# Autodesk Inventor assembly: крепление
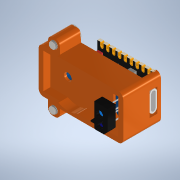
[picture p0: Inventor's stored thumbnail of the model, 180x180]
Saved by Autodesk Inventor 2022 (Build 260153000, 153)
## iProperties
Created: 2025-02-02
Part Number: крепление
Document SubType Name: Assembly
Designer: Admin
Author: Admin
## Documents named in this file (5)
- G:\машина\крепление.iam
- G:\машина\крепл. датчк.1.ipt
- G:\машина\ESP32S3 Super Mini.ipt
- G:\машина\Screw GB_T 13806.1-1992 B M3 x 10.ipt
- G:\машина\TCRT5000.iam
## Components (5 placed, 4 different names)
1. крепл. датчк.1:1 — Совмещение:7
2. ESP32S3 Super Mini:1
3. Screw GB/T 13806.1-1992 Type B M3 x 10:1 — Совмещение:7
4. Screw GB/T 13806.1-1992 Type B M3 x 10:2
5. TCRT5000:1 [sub-assembly]
## Relationships (10: Mate 6, Flush 4)
- [Mate]: крепл. датчк.1:1 ↔ ESP32S3 Super Mini:1
- [Flush]: крепл. датчк.1:1 ↔ ESP32S3 Super Mini:1
- [Flush]: крепл. датчк.1:1 ↔ ESP32S3 Super Mini:1
- [Mate]: крепл. датчк.1:1 ↔ Screw GB/T 13806.1-1992 Type B M3 x 10:2
- [Flush]: крепл. датчк.1:1 ↔ Screw GB/T 13806.1-1992 Type B M3 x 10:2
- [Flush]: крепл. датчк.1:1 ↔ Screw GB/T 13806.1-1992 Type B M3 x 10:1
- [Mate]: крепл. датчк.1:1 ↔ TCRT5000:1
- [Mate]: крепл. датчк.1:1 ↔ TCRT5000:1
- [Mate]: крепл. датчк.1:1 ↔ TCRT5000:1
- Совмещение:7 [Mate]: крепл. датчк.1:1 ↔ Screw GB/T 13806.1-1992 Type B M3 x 10:1
